# Autodesk Inventor assembly: Attachment
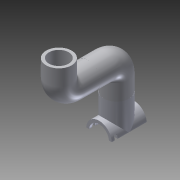
[picture p0: Inventor's stored thumbnail of the model, 180x180]
Saved by Autodesk Inventor 2013 (Build 170138000, 138)
## iProperties
Created: 2014-08-06
Part Number: Attachment
Document SubType Name: Assembly
Designer: Kyle
Author: Kyle
## Documents named in this file (4)
- C:\Users\Kyle\Documents\Autodesk\Inventor\Projects\ROV\Arm\Attachment.iam
- C:\Users\Kyle\Documents\Autodesk\Inventor\Projects\ROV\Arm\0.5 Frame Mount.ipt
- C:\Users\Kyle\Documents\Autodesk\Inventor\Projects\ROV\Arm\Flush Connect Pipe.ipt
- C:\Users\Kyle\Documents\Autodesk\Inventor\Projects\ROV\Arm\0.5 Elbow.ipt
## Components (5 placed, 3 different names)
1. 0.5 Frame Mount:1 — Mate:1, Mate:2, Mate:4, Angle:1, Angle:2
2. Flush Connect Pipe:1 — Mate:1, Mate:2, Mate:3
3. 0.5 Elbow:1 — Mate:3, Mate:4, Angle:1, Mate:5, Mate:6, Mate:8
4. Flush Connect Pipe:2 — Mate:5, Mate:6, Mate:7
5. 0.5 Elbow:2 — Mate:7, Angle:2, Mate:8
## Relationships (10: Mate 8, Angle 2)
- Mate:1: 0.5 Frame Mount:1 ↔ Flush Connect Pipe:1
- Mate:2: 0.5 Frame Mount:1 ↔ Flush Connect Pipe:1
- Mate:3: Flush Connect Pipe:1 ↔ 0.5 Elbow:1
- Mate:4: 0.5 Frame Mount:1 ↔ 0.5 Elbow:1
- Angle:1 (0 deg): 0.5 Frame Mount:1 ↔ 0.5 Elbow:1
- Mate:5: 0.5 Elbow:1 ↔ Flush Connect Pipe:2
- Mate:6: 0.5 Elbow:1 ↔ Flush Connect Pipe:2
- Mate:7: Flush Connect Pipe:2 ↔ 0.5 Elbow:2
- Angle:2 (180 deg): 0.5 Frame Mount:1 ↔ 0.5 Elbow:2
- Mate:8: 0.5 Elbow:1 ↔ 0.5 Elbow:2
